# Autodesk Inventor assembly: Eye_Assemble
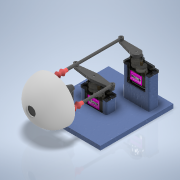
[picture p0: Inventor's stored thumbnail of the model, 180x180]
Saved by Autodesk Inventor 2022 (Build 260153000, 153)
## iProperties
Created: 2021-11-09
Part Number: Eye_Assemble
Document SubType Name: Assembly
Designer: Juan
Author: Juan
## Documents named in this file (14)
- C:\Users\Juan\Documents\3D Printer Models\Eye_Assemble.iam
- C:\Users\Juan\Documents\3D Printer Models\Camera.ipt
- C:\Users\Juan\Documents\3D Printer Models\Eye.ipt
- C:\Users\Juan\Documents\3D Printer Models\Pin.ipt
- C:\Users\Juan\Documents\3D Printer Models\Flex.ipt
- C:\Users\Juan\Documents\3D Printer Models\Ball.ipt
- C:\Users\Juan\Documents\3D Printer Models\BallFemale.ipt
- C:\Users\Juan\Documents\3D Printer Models\BarX40mm.ipt
- C:\Users\Juan\Documents\3D Printer Models\ServoXAxis.ipt
- C:\Users\Juan\Downloads\mg90s-servo-high-detail-1.snapshot.49\inventor files(shrinkwrap)\Assembly SERVO.iam
- C:\Users\Juan\Documents\3D Printer Models\BarX70mm.ipt
- C:\Users\Juan\Documents\3D Printer Models\ServoYAxis.ipt
- C:\Users\Juan\Documents\3D Printer Models\Base.ipt
- C:\Users\caspe\Downloads\20210119_143510.jpg
## Components (18 placed, 12 different names)
1. Base:1 — Insert:1, Insert:2, Mate:1, Mate:2, Mate:3, Flush:1, Flush:2
2. BallFemale:1 — Insert:1, Insert:2, Ball:1
3. Eye:1 — Insert:3, Insert:4, Insert:5, Insert:6, Insert:7
4. Camera:1 — Insert:3
5. Pin:1 — Insert:4, Insert:9
6. Pin:2 — Insert:5, Insert:8
7. Pin:3 — Insert:6, Insert:10
8. Ball:2 — Insert:7, Ball:1
9. Flex:1 — Insert:9, Insert:17, Mate:4
10. Flex:2 — Insert:8, Insert:14
11. Flex:3 — Insert:10, Insert:15
12. Assembly SERVO:1 [sub-assembly] — Mate:1, Mate:2, Insert:11
13. ServoXAxis:1 — Insert:11, Insert:12, Insert:13
14. BarX40mm:1 — Insert:13, Insert:14
15. BarX40mm:2 — Insert:12, Insert:15
16. Assembly SERVO:2 [sub-assembly] — Mate:3, Flush:1, Flush:2, Insert:16
17. ServoYAxis:1 — Insert:16, Rigid:1
18. BarX70mm:1 — Insert:17, Rigid:1, Mate:4
## Relationships (25: Insert 17, Mate 4, Flush 2, BallJoint 1, WeldJoint 1)
- Insert:1: Base:1 ↔ BallFemale:1
- Insert:2: Base:1 ↔ BallFemale:1
- Insert:3: Eye:1 ↔ Camera:1
- Insert:4: Eye:1 ↔ Pin:1
- Insert:5: Eye:1 ↔ Pin:2
- Insert:6: Eye:1 ↔ Pin:3
- Insert:7: Eye:1 ↔ Ball:2
- Ball:1: BallFemale:1 ↔ Ball:2
- Insert:8: Pin:2 ↔ Flex:2
- Insert:9: Pin:1 ↔ Flex:1
- Insert:10: Pin:3 ↔ Flex:3
- Mate:1: Base:1 ↔ Assembly SERVO:1
- Mate:2: Base:1 ↔ Assembly SERVO:1
- Insert:11: Assembly SERVO:1 ↔ ServoXAxis:1
- Insert:12: ServoXAxis:1 ↔ BarX40mm:2
- Insert:13: ServoXAxis:1 ↔ BarX40mm:1
- Insert:14: Flex:2 ↔ BarX40mm:1
- Insert:15: Flex:3 ↔ BarX40mm:2
- Mate:3: Base:1 ↔ Assembly SERVO:2
- Flush:1: Base:1 ↔ Assembly SERVO:2
- Flush:2: Base:1 ↔ Assembly SERVO:2
- Insert:16: Assembly SERVO:2 ↔ ServoYAxis:1
- Insert:17: Flex:1 ↔ BarX70mm:1
- Rigid:1 [WeldJoint]: ServoYAxis:1 ↔ BarX70mm:1
- Mate:4: Flex:1 ↔ BarX70mm:1
